# Autodesk Inventor assembly: leg_bone_1
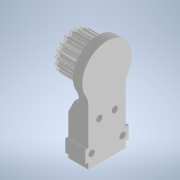
[picture p0: Inventor's stored thumbnail of the model, 180x180]
Saved by Autodesk Inventor 2020 (Build 240168000, 168)
## iProperties
Created: 2019-05-02
Part Number: leg_bone_1
Document SubType Name: Assembly
Designer: psrob
Author: psrob
## Documents named in this file (3)
- E:\projects-2\project dog gen2\hardware\leg_bone_1.iam
- E:\projects-2\project dog gen2\hardware\leg_bone_2.ipt
- E:\projects-2\project dog gen2\hardware\GT2_20T_2.ipt
## Components (2 placed, 2 different names)
1. leg_bone_2:1 — Insert:1
2. GT2_20T_2:1 — Insert:1
## Relationships (1: Insert 1)
- Insert:1: leg_bone_2:1 ↔ GT2_20T_2:1
